# Autodesk Inventor assembly: 3 Flex, LS
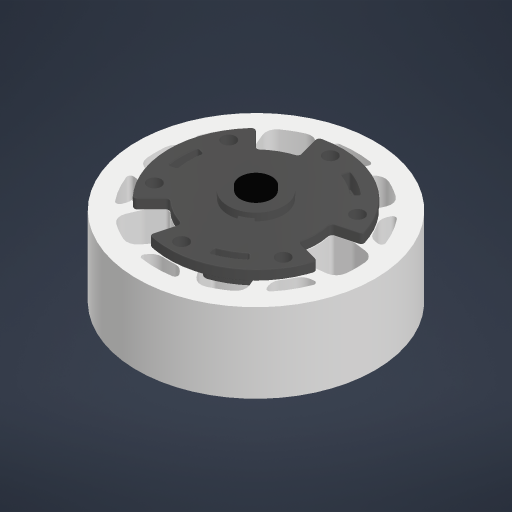
[picture p0: Inventor's stored thumbnail of the model, 512x512]
Saved by Autodesk Inventor 2023 (Build 270158000, 158)
## iProperties
Created: 2023-02-19
Part Number: 3 Flex, LS
Document SubType Name: Assembly
Designer: Windows Macbook
Author: Windows Macbook
## Documents named in this file (6)
- C:\Users\Windows Macbook\Desktop\Inventor\Motion\Wheels\Flex Wheels\3 Flex, LS.iam
- C:\Users\Windows Macbook\Desktop\Inventor\Motion\Wheels\Flex Wheels\3.000 Flex Wheel\3.000 30A 1.000.ipt
- C:\Users\Windows Macbook\Desktop\Inventor\Motion\Wheels\Flex Wheels\3.000 Flex Wheel.ipt
- C:\Users\Windows Macbook\Desktop\Inventor\Motion\Wheels\Flex Wheels\VersaHub.ipt
- C:\Users\Windows Macbook\Desktop\Inventor\Motion\Wheels\Flex Wheels\VersaHex Adapters .250.ipt
- C:\Users\Windows Macbook\Desktop\Inventor\Motion\Insert Square.ipt
## Components (7 placed, 4 different names)
1. 3.000 30A 1.000:1 — Insert:5, Insert:6, Insert:7, Insert:8
2. VersaHub:1 — Insert:7, Insert:8
3. VersaHex Adapters .250:1
4. Insert Square:1
5. VersaHub:2 — Insert:5, Insert:6
6. VersaHex Adapters .250:2
7. Insert Square:2
## Relationships (12: Insert 8, Angle 2, Mate 2)
- [Insert]: VersaHex Adapters .250:1 ↔ Insert Square:1
- [Angle] (0 deg): VersaHex Adapters .250:1 ↔ Insert Square:1
- [Insert]: VersaHub:1 ↔ VersaHex Adapters .250:1
- [Mate]: VersaHub:1 ↔ VersaHex Adapters .250:1
- [Insert]: VersaHex Adapters .250:2 ↔ Insert Square:2
- [Angle] (0 deg): VersaHex Adapters .250:2 ↔ Insert Square:2
- [Insert]: VersaHub:2 ↔ VersaHex Adapters .250:2
- [Mate]: VersaHub:2 ↔ VersaHex Adapters .250:2
- Insert:5: 3.000 30A 1.000:1 ↔ VersaHub:2
- Insert:6: 3.000 30A 1.000:1 ↔ VersaHub:2
- Insert:7: 3.000 30A 1.000:1 ↔ VersaHub:1
- Insert:8: 3.000 30A 1.000:1 ↔ VersaHub:1
## Named parameters: d8_d0 = 0 mm, d9_d1 = 0 deg, d10_d2 = 0 mm, d11_d5 = 0 mm
